# Autodesk Inventor assembly: 하단부 조립품
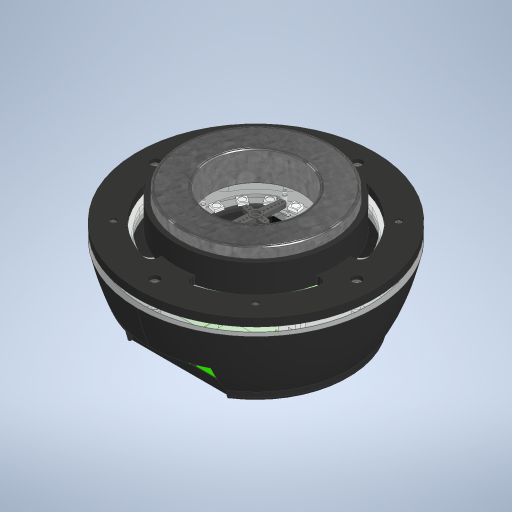
[picture p0: Inventor's stored thumbnail of the model, 512x512]
Saved by Autodesk Inventor 2023 (Build 270158000, 158)
## iProperties
Created: 2022-06-02
Part Number: 하단부 조립품
Document SubType Name: Assembly
Designer: fly01
Author: fly01
## Documents named in this file (10)
- C:\Users\fly01\Desktop\2022카이스트 입학준비\스마트홈\제작부품'\하단부 조립품.iam
- C:\Users\fly01\Desktop\2022카이스트 입학준비\스마트홈\제작부품'\메인 형상_하단.ipt
- C:\Users\fly01\Desktop\2022카이스트 입학준비\스마트홈\범용 부품\raspberry.ipt
- C:\Users\fly01\Desktop\2022카이스트 입학준비\스마트홈\범용 부품\육각렌치볼트 m3 15mm.ipt
- C:\Users\fly01\Desktop\2022카이스트 입학준비\스마트홈\제작부품'\하단부 뚜껑.iam
- C:\Users\fly01\Desktop\2022카이스트 입학준비\스마트홈\범용 부품\십자 둥근머리 볼트 6mm.ipt
- C:\Users\fly01\Desktop\2022카이스트 입학준비\스마트홈\제작부품'\하단 맨 위부분.ipt
- C:\Users\fly01\Desktop\2022카이스트 입학준비\스마트홈\범용 부품\180도 서보모터 십자축.ipt
- C:\Users\fly01\Desktop\2022카이스트 입학준비\스마트홈\제작부품'\스피커 조립부품.ipt
- C:\Users\fly01\Desktop\2022카이스트 입학준비\스마트홈\범용 부품\6011베어링.ipt
## Components (21 placed, 9 different names)
1. 메인 형상_하단:1 — 회전:1, 삽입:1, 삽입:11, 강체:1
2. raspberry:1 — 회전:1, 삽입:1, 삽입:7, 삽입:8, 삽입:9, 삽입:10
3. 육각렌치볼트 m3 15mm:1 — 삽입:13, 삽입:16
4. 육각렌치볼트 m3 15mm:2 — 삽입:12
5. 육각렌치볼트 m3 15mm:3 — 삽입:15, 삽입:17
6. 육각렌치볼트 m3 15mm:4 — 삽입:14
7. 십자 둥근머리 볼트 6mm:1 — 삽입:7
8. 십자 둥근머리 볼트 6mm:2 — 삽입:10
9. 십자 둥근머리 볼트 6mm:3 — 삽입:8
10. 십자 둥근머리 볼트 6mm:4 — 삽입:9
11. 하단부 뚜껑:1 [sub-assembly] — 삽입:11, 삽입:12, 삽입:13, 삽입:14, 삽입:15, 삽입:25
12. 하단 맨 위부분:1 — 삽입:16, 삽입:17, 삽입:18, 삽입:19, 삽입:20, 삽입:21, 회전:2
13. 십자 둥근머리 볼트 6mm:5 — 삽입:21
14. 십자 둥근머리 볼트 6mm:6 — 삽입:20
15. 십자 둥근머리 볼트 6mm:7 — 삽입:18
16. 십자 둥근머리 볼트 6mm:8 — 삽입:19
17. 180도 서보모터 십자축:1 — 삽입:25
18. 스피커 조립부품:1 — 강체:1, 삽입:23, 삽입:24
19. 십자 둥근머리 볼트 6mm:9 — 삽입:24
20. 십자 둥근머리 볼트 6mm:10 — 삽입:23
21. 6011베어링:1 — 회전:2
## Relationships (22: Insert 19, RevoluteJoint 2, WeldJoint 1)
- 회전:1 [RevoluteJoint]: 메인 형상_하단:1 ↔ raspberry:1
- 삽입:1 [Insert]: 메인 형상_하단:1 ↔ raspberry:1
- 삽입:7 [Insert]: raspberry:1 ↔ 십자 둥근머리 볼트 6mm:1
- 삽입:8 [Insert]: raspberry:1 ↔ 십자 둥근머리 볼트 6mm:3
- 삽입:9 [Insert]: raspberry:1 ↔ 십자 둥근머리 볼트 6mm:4
- 삽입:10 [Insert]: raspberry:1 ↔ 십자 둥근머리 볼트 6mm:2
- 삽입:11 [Insert] (0.2 mm): 메인 형상_하단:1 ↔ 하단부 뚜껑:1
- 삽입:12 [Insert]: 육각렌치볼트 m3 15mm:2 ↔ 하단부 뚜껑:1
- 삽입:13 [Insert]: 육각렌치볼트 m3 15mm:1 ↔ 하단부 뚜껑:1
- 삽입:14 [Insert]: 육각렌치볼트 m3 15mm:4 ↔ 하단부 뚜껑:1
- 삽입:15 [Insert]: 육각렌치볼트 m3 15mm:3 ↔ 하단부 뚜껑:1
- 삽입:16 [Insert]: 육각렌치볼트 m3 15mm:1 ↔ 하단 맨 위부분:1
- 삽입:17 [Insert]: 육각렌치볼트 m3 15mm:3 ↔ 하단 맨 위부분:1
- 삽입:18 [Insert]: 하단 맨 위부분:1 ↔ 십자 둥근머리 볼트 6mm:7
- 삽입:19 [Insert]: 하단 맨 위부분:1 ↔ 십자 둥근머리 볼트 6mm:8
- 삽입:20 [Insert]: 하단 맨 위부분:1 ↔ 십자 둥근머리 볼트 6mm:6
- 삽입:21 [Insert]: 하단 맨 위부분:1 ↔ 십자 둥근머리 볼트 6mm:5
- 강체:1 [WeldJoint]: 메인 형상_하단:1 ↔ 스피커 조립부품:1
- 삽입:23 [Insert]: 스피커 조립부품:1 ↔ 십자 둥근머리 볼트 6mm:10
- 삽입:24 [Insert]: 스피커 조립부품:1 ↔ 십자 둥근머리 볼트 6mm:9
- 삽입:25 [Insert]: 하단부 뚜껑:1 ↔ 180도 서보모터 십자축:1
- 회전:2 [RevoluteJoint]: 하단 맨 위부분:1 ↔ 6011베어링:1
